# Autodesk Inventor assembly: club_ABS_all
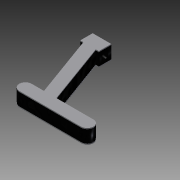
[picture p0: Inventor's stored thumbnail of the model, 180x180]
Saved by Autodesk Inventor 2015 SP1 (Build 190203100, 203)
## iProperties
Created: 2015-03-24
Part Number: club_ABS_all
Document SubType Name: Assembly
Designer: Marcin
Author: Marcin
## Documents named in this file (3)
- C:\Users\Marcin\Documents\Inventor\SynerGolf\club\club_ABS_all.iam
- C:\Users\Marcin\Documents\Inventor\SynerGolf\club\club_ABS.ipt
- C:\Users\Marcin\Documents\Inventor\SynerGolf\club\club_ABS_metal.ipt
## Components (3 placed, 2 different names)
1. club_ABS:1 — Równoległy:1, Równoległy:2, Równoległy:3, Równoległy:4, Równoległy:5, Zestawiający:1, Zestawiający:2, Zestawiający:3
2. club_ABS_metal:1 — Równoległy:4, Równoległy:5
3. club_ABS_metal:2 — Zestawiający:1, Zestawiający:2, Zestawiający:3
## Relationships (8: Flush 5, Mate 3)
- Równoległy:1 [Flush]: club_ABS:1
- Równoległy:2 [Flush]: club_ABS:1
- Równoległy:3 [Flush]: club_ABS:1
- Równoległy:4 [Flush]: club_ABS:1 ↔ club_ABS_metal:1
- Równoległy:5 [Flush]: club_ABS:1 ↔ club_ABS_metal:1
- Zestawiający:1 [Mate]: club_ABS:1 ↔ club_ABS_metal:2
- Zestawiający:2 [Mate]: club_ABS:1 ↔ club_ABS_metal:2
- Zestawiający:3 [Mate]: club_ABS:1 ↔ club_ABS_metal:2
